# Autodesk Inventor assembly: IndexBeltSys
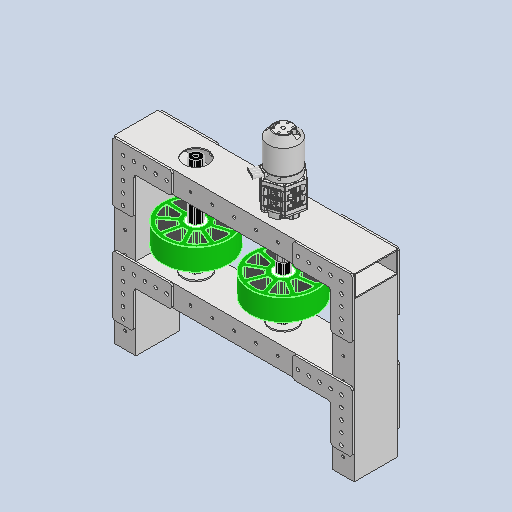
[picture p0: Inventor's stored thumbnail of the model, 512x512]
Saved by Autodesk Inventor 2022 (Build 260153000, 153)
## iProperties
Created: 2022-01-13
Part Number: IndexBeltSys
Document SubType Name: Assembly
Designer: tagaz
Author: tagaz
## Documents named in this file (12)
- C:\Users\tagaz\OneDrive\Documents\T3-Cad\CAD\2022 Parts\Index\IndexBeltSys.iam
- IndexSys.iam
- C:\Users\tagaz\OneDrive\Documents\T3-Cad\CAD\2022 Parts\Generic\VersaFrame_IndexSupp.ipt
- C:\Users\tagaz\OneDrive\Documents\T3-Cad\CAD\2022 Parts\Generic\VersaFrame_VelcRail.ipt
- C:\Users\tagaz\OneDrive\Documents\T3-Cad\CAD\Generic and Stock\VersaGusset 90o.ipt
- C:\Users\tagaz\OneDrive\Documents\T3-Cad\CAD\Bearing  for THUNDER.ipt
- C:\Users\tagaz\OneDrive\Documents\T3-Cad\CAD\2022 Parts\Generic\VersaFrame_VelcRail2.ipt
- C:\Users\tagaz\OneDrive\Documents\T3-Cad\CAD\2022 Parts\Generic\indexThundershaft.ipt
- C:\Users\tagaz\OneDrive\Documents\T3-Cad\CAD\2022 Parts\Generic\indexThundershaft2.ipt
- C:\Users\tagaz\OneDrive\Documents\T3-Cad\CAD\2022 Parts\Generic\16T Alum Hub Sprock 25 Chain.ipt
- C:\Users\tagaz\OneDrive\Documents\T3-Cad\CAD\2022 Parts\Generic\3in Compliance wheel.ipt
- C:\Users\tagaz\OneDrive\Documents\T3-Cad\CAD\Generic and Stock\RevMotorParts\Neo550Assembly.iam
## Components (25 placed, 10 different names)
1. VersaFrame_IndexSupp:1 — Flush:5, Flush:6, Mate:3, Flush:8, Flush:9, Flush:24, Mate:31, Flush:55, Flush:56
2. VersaFrame_IndexSupp:2 — Mate:2, Flush:3, Flush:4, Mate:6, Flush:12, Mate:7
3. VersaFrame_VelcRail:1 — Mate:2, Flush:3, Flush:4, Flush:5, Flush:6, Mate:3, Flush:7, Mate:4, Mate:5, Flush:10, Flush:11, Flush:13, Flush:14, Insert:2, Insert:3, Mate:30, Mate:59, Mate:60
4. Bearing  for THUNDER:1 — Insert:3
5. Bearing  for THUNDER:2 — Insert:2
6. Bearing  for THUNDER:7 — Insert:6
7. Bearing  for THUNDER:8 — Insert:7, Mate:56, Mate:57
8. VersaFrame_VelcRail2:1 — Flush:24, Mate:30, Mate:31, Insert:6, Insert:7, Insert:8, Insert:9
9. Bearing  for THUNDER:9 — Insert:9, Mate:62
10. Bearing  for THUNDER:10 — Insert:8
11. 16T Alum Hub Sprock 25 Chain:4
12. 16T Alum Hub Sprock 25 Chain:5
13. 3in Compliance wheel:1 — Flush:56, Mate:65, Mate:66
14. 3in Compliance wheel:2 — Flush:55, Mate:63, Mate:64
15. indexThundershaft:3 — Mate:56, Mate:57, Mate:65, Mate:66
16. Neo550Assembly:1 [sub-assembly] — Mate:59, Mate:60, Mate:61, Flush:57, Flush:58
17. indexThundershaft2:1 — Mate:61, Flush:57, Flush:58, Mate:62, Mate:63, Mate:64
18. VersaGusset 90o:4 — Mate:6, Flush:11, Flush:12
19. VersaGusset 90o:3 — Mate:7, Flush:13, Flush:14
20. VersaGusset 90o:1 — Mate:5, Flush:9, Flush:10
21. VersaGusset 90o:2 — Flush:7, Mate:4, Flush:8
22. VersaGusset 90o:5
23. VersaGusset 90o:6
24. VersaGusset 90o:7
25. VersaGusset 90o:8
## Component patterns: (2 elements, first: VersaGusset 90o:4 + VersaGusset 90o:3 + VersaGusset 90o:1 + VersaGusset 90o:2)
## Relationships (41: Mate 18, Flush 17, Insert 6)
- Mate:2: VersaFrame_IndexSupp:2 ↔ VersaFrame_VelcRail:1
- Flush:3: VersaFrame_IndexSupp:2 ↔ VersaFrame_VelcRail:1
- Flush:4: VersaFrame_IndexSupp:2 ↔ VersaFrame_VelcRail:1
- Flush:5: VersaFrame_IndexSupp:1 ↔ VersaFrame_VelcRail:1
- Flush:6: VersaFrame_IndexSupp:1 ↔ VersaFrame_VelcRail:1
- Mate:3: VersaFrame_IndexSupp:1 ↔ VersaFrame_VelcRail:1
- Flush:7: VersaFrame_VelcRail:1 ↔ VersaGusset 90o:2
- Mate:4: VersaFrame_VelcRail:1 ↔ VersaGusset 90o:2
- Flush:8: VersaFrame_IndexSupp:1 ↔ VersaGusset 90o:2
- Mate:5: VersaFrame_VelcRail:1 ↔ VersaGusset 90o:1
- Flush:9: VersaFrame_IndexSupp:1 ↔ VersaGusset 90o:1
- Flush:10: VersaFrame_VelcRail:1 ↔ VersaGusset 90o:1
- Mate:6: VersaFrame_IndexSupp:2 ↔ VersaGusset 90o:4
- Flush:11: VersaFrame_VelcRail:1 ↔ VersaGusset 90o:4
- Flush:12: VersaFrame_IndexSupp:2 ↔ VersaGusset 90o:4
- Mate:7: VersaFrame_IndexSupp:2 ↔ VersaGusset 90o:3
- Flush:13: VersaFrame_VelcRail:1 ↔ VersaGusset 90o:3
- Flush:14: VersaFrame_VelcRail:1 ↔ VersaGusset 90o:3
- Insert:2: VersaFrame_VelcRail:1 ↔ Bearing  for THUNDER:2
- Insert:3: VersaFrame_VelcRail:1 ↔ Bearing  for THUNDER:1
- Flush:24: VersaFrame_IndexSupp:1 ↔ VersaFrame_VelcRail2:1
- Mate:30 (88.9 mm): VersaFrame_VelcRail:1 ↔ VersaFrame_VelcRail2:1
- Mate:31: VersaFrame_IndexSupp:1 ↔ VersaFrame_VelcRail2:1
- Insert:6: Bearing  for THUNDER:7 ↔ VersaFrame_VelcRail2:1
- Insert:7: Bearing  for THUNDER:8 ↔ VersaFrame_VelcRail2:1
- Insert:8: VersaFrame_VelcRail2:1 ↔ Bearing  for THUNDER:10
- Insert:9: VersaFrame_VelcRail2:1 ↔ Bearing  for THUNDER:9
- Flush:55 (120.65 mm): VersaFrame_IndexSupp:1 ↔ 3in Compliance wheel:2
- Flush:56 (-120.65 mm): VersaFrame_IndexSupp:1 ↔ 3in Compliance wheel:1
- Mate:56: Bearing  for THUNDER:8 ↔ indexThundershaft:3
- Mate:57: Bearing  for THUNDER:8 ↔ indexThundershaft:3
- Mate:59: VersaFrame_VelcRail:1 ↔ Neo550Assembly:1
- Mate:60: VersaFrame_VelcRail:1 ↔ Neo550Assembly:1
- Mate:61: Neo550Assembly:1 ↔ indexThundershaft2:1
- Flush:57: Neo550Assembly:1 ↔ indexThundershaft2:1
- Flush:58: Neo550Assembly:1 ↔ indexThundershaft2:1
- Mate:62: Bearing  for THUNDER:9 ↔ indexThundershaft2:1
- Mate:63: 3in Compliance wheel:2 ↔ indexThundershaft2:1
- Mate:64: 3in Compliance wheel:2 ↔ indexThundershaft2:1
- Mate:65: 3in Compliance wheel:1 ↔ indexThundershaft:3
- Mate:66: 3in Compliance wheel:1 ↔ indexThundershaft:3
